# Autodesk Inventor assembly: car_2
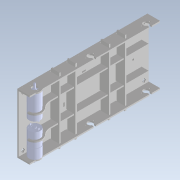
[picture p0: Inventor's stored thumbnail of the model, 180x180]
Saved by Autodesk Inventor 2022 (Build 260153000, 153)
## iProperties
Created: 2023-04-28
Part Number: car_2
Document SubType Name: Assembly
Designer: Johnny Jou
Author: Johnny Jou
## Documents named in this file (6)
- C:\Users\JOU\Desktop\git\Areo_Rider_Cabin\car\car_2.iam
- C:\Users\JOU\Desktop\git\Areo_Rider_Cabin\car\chassis_1_1_3.ipt
- C:\Users\JOU\Desktop\git\Areo_Rider_Cabin\car\外抓檔\25GA370.ipt
- C:\Users\JOU\Desktop\git\Areo_Rider_Cabin\car\chassis_1_5.ipt
- C:\Users\JOU\Desktop\git\Areo_Rider_Cabin\car\chassis_1_6.ipt
- C:\Users\JOU\Desktop\git\Areo_Rider_Cabin\car\plate_2.ipt
## Components (11 placed, 5 different names)
1. chassis_1_1_3:1 — 貼合:1, 貼合:2, 貼合:3, 齊平:1, 貼合:11, 貼合:12, 貼合:22, 貼合:23
2. chassis_1_1_3:2 — 貼合:4, 貼合:5, 貼合:6, 齊平:1, 貼合:10, 貼合:21
3. 25GA370:1 — 貼合:1, 貼合:2, 貼合:3, 貼合:7, 貼合:9
4. 25GA370:2 — 貼合:4, 貼合:5, 貼合:6, 貼合:7, 貼合:8
5. chassis_1_5:1 — 貼合:9, 齊平:5, 貼合:11, 齊平:10, 齊平:11, 齊平:12, 齊平:13, 貼合:13, 貼合:14
6. chassis_1_5:2 — 貼合:8, 齊平:5, 貼合:10, 貼合:15, 貼合:16, 貼合:17, 貼合:18, 貼合:19, 貼合:20
7. chassis_1_6:1 — 齊平:7, 齊平:8, 齊平:9, 齊平:13, 貼合:13, 貼合:14
8. chassis_1_6:2 — 齊平:8, 貼合:12, 齊平:10, 貼合:17, 貼合:18
9. chassis_1_6:3 — 齊平:9, 齊平:11, 貼合:19, 貼合:20
10. chassis_1_6:4 — 齊平:7, 齊平:12, 貼合:15, 貼合:16
11. plate_2:1 — 貼合:21, 貼合:22, 貼合:23
## Relationships (32: Mate 23, Flush 9)
- 貼合:1 [Mate]: chassis_1_1_3:1 ↔ 25GA370:1
- 貼合:2 [Mate]: chassis_1_1_3:1 ↔ 25GA370:1
- 貼合:3 [Mate]: chassis_1_1_3:1 ↔ 25GA370:1
- 貼合:4 [Mate]: chassis_1_1_3:2 ↔ 25GA370:2
- 貼合:5 [Mate]: chassis_1_1_3:2 ↔ 25GA370:2
- 貼合:6 [Mate]: chassis_1_1_3:2 ↔ 25GA370:2
- 齊平:1 [Flush]: chassis_1_1_3:1 ↔ chassis_1_1_3:2
- 貼合:7 [Mate] (20 mm): 25GA370:1 ↔ 25GA370:2
- 貼合:8 [Mate]: 25GA370:2 ↔ chassis_1_5:2
- 貼合:9 [Mate]: 25GA370:1 ↔ chassis_1_5:1
- 齊平:5 [Flush]: chassis_1_5:1 ↔ chassis_1_5:2
- 貼合:10 [Mate] (35 mm): chassis_1_1_3:2 ↔ chassis_1_5:2
- 貼合:11 [Mate] (35 mm): chassis_1_1_3:1 ↔ chassis_1_5:1
- 齊平:7 [Flush]: chassis_1_6:1 ↔ chassis_1_6:4
- 齊平:8 [Flush]: chassis_1_6:1 ↔ chassis_1_6:2
- 齊平:9 [Flush]: chassis_1_6:1 ↔ chassis_1_6:3
- 貼合:12 [Mate]: chassis_1_1_3:1 ↔ chassis_1_6:2
- 齊平:10 [Flush]: chassis_1_5:1 ↔ chassis_1_6:2
- 齊平:11 [Flush]: chassis_1_5:1 ↔ chassis_1_6:3
- 齊平:12 [Flush]: chassis_1_5:1 ↔ chassis_1_6:4
- 齊平:13 [Flush]: chassis_1_5:1 ↔ chassis_1_6:1
- 貼合:13 [Mate]: chassis_1_5:1 ↔ chassis_1_6:1
- 貼合:14 [Mate]: chassis_1_5:1 ↔ chassis_1_6:1
- 貼合:15 [Mate]: chassis_1_5:2 ↔ chassis_1_6:4
- 貼合:16 [Mate]: chassis_1_5:2 ↔ chassis_1_6:4
- 貼合:17 [Mate]: chassis_1_5:2 ↔ chassis_1_6:2
- 貼合:18 [Mate]: chassis_1_5:2 ↔ chassis_1_6:2
- 貼合:19 [Mate]: chassis_1_5:2 ↔ chassis_1_6:3
- 貼合:20 [Mate]: chassis_1_5:2 ↔ chassis_1_6:3
- 貼合:21 [Mate]: chassis_1_1_3:2 ↔ plate_2:1
- 貼合:22 [Mate]: chassis_1_1_3:1 ↔ plate_2:1
- 貼合:23 [Mate]: chassis_1_1_3:1 ↔ plate_2:1
